# Autodesk Inventor assembly: 041.5
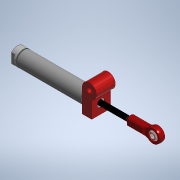
[picture p0: Inventor's stored thumbnail of the model, 180x180]
Saved by Autodesk Inventor 2020 (Build 240168000, 168)
## iProperties
Part Number: 041.5
Catalog Web Link: www.cadenas.de
Description: Original Line Standard Air Cylinders-Standard Air Cylinders
Vendor: BIMBA
Document SubType Name: Assembly
Designer: partserver
Manufacturer: BIMBA
Mass: 46.5963 g
Surface Area: 273.014 cm^2
Volume: 39.6045 cm^3
Density: 1.17654 g/cm^3
Category: PARTsolutions
Company: BIMBA
PSOL_IDENT_0: {$CADENAS_DATA\23d-libs\bimba\bimba_brand\bimba_imperial\bimba_full_line\original_line_cylinders\sta
PSOL_IDENT_1: ndard_air_cylinders\standard_air_cylinder_asmtab.prj},318 {VTYP=3D},{STYP=ASSTAB},{NB=041.5},{LINA=0
PSOL_IDENT_2: 41.5},{NN=Original Line Standard Air Cylinders},{DATE=19.01.2022 10:19:38},{GEOMDATE=11.11.2021 07:3
PSOL_IDENT_3: 1:43},{VERSION=},{LINEID=50},{WBVAR=STROKE,ACTING,MNT,DER,NR,BM,CO,OO,VO,M,EE,EEL,K,Q,Y,G,T,HL,B,H,S
PSOL_IDENT_4: ER,SR,NT,W,STPT1,STPT2,STPT3,STPT4,MB,PB,PRC,TB,MN},{WBNUMERIC=STROKE,EEL}  {NB=041.5},{LINA=041.5},
PSOL_IDENT_5: {KT=DUMMY},{PN=041.5},{PNC=041.5},{PNA=(NO ACCESSORIES)},{PNAHELP=},{DASH=},{BORE1=0.75000000},{BORE=
PSOL_IDENT_6: 3/4\" (04)},{BOREPN=04},{STROKE=1.500},{STROKEALG=[0.011:50/0.001]},{STROKE1=1.500},{ACTING=},{ACTIN
PSOL_IDENT_7: GALG= '' , 'Single Acting' , 'R' , 'Reverse Single Acting (R)' , 'D' , 'Double Acting (D)' },{ACTING
PSOL_IDENT_8: PN=},{MNT=},{MNTALG= '' , 'Front Nose Mounting' , 'P' , 'Rear Pivot Mounting (P)' , 'BF' , 'Front Bl
PSOL_IDENT_9: ock Mounting (BF)' , 'BR' , 'Rear Block Mounting for Vertical Positioning (BR)' , 'BFT' , 'Front Blo
PSOL_IDENT_10: ck Trunnion Mounting (BFT)' , 'BRT' , 'Rear Block Trunnion Mounting (BRT)' , 'A' , 'Double End Mount
PSOL_IDENT_11: ing with Brackets and Adjustable Stroke (A)' , 'AP' , 'Rear Pivot Mounting with Adjustable Stroke (A
PSOL_IDENT_12: P)' },{TYPE=},{MNTPN=},{DER=},{DERALG= '' , 'N/A' },{NR=},{NRALG= '' , 'Round (Standard)' , 'NR' , '
PSOL_IDENT_13: Non-rotating - Hexagon Rod' },{NRPN=},{BM=},{BMALG= '' , 'Without Built-in Midget 3-Way Solenoid Ope
PSOL_IDENT_14: rated Valve' , 'LS' , 'With LS Series Solenoid Valve [LS]' },{BMPN=},{CO=},{COALG= '' , 'N/A' },{OO=
PSOL_IDENT_15: },{OOALG= '', 'N/A' },{OOPN=},{VO=Z},{VOALG= 'Z' , 'N/A' },{VOPN=},{OOVOPN=},{M=},{MALG= '', 'Withou
PSOL_IDENT_16: t Magnet', 'M', 'With Magnet' },{EE=},{EEL=0.000},{EEMAX=48.5000},{EEALG= '', 'Without Extra Extensi
PSOL_IDENT_17: on', 'EE', 'With Extra Extension' },{EELALG=0},{EEPN=},{EEPN1=0.000},{K=},{KALG= '' , 'N/A' },{KPN=}
PSOL_IDENT_18: ,{Q=},{QALG= '' , 'Standard Port' , 'Q' , 'Side Port' },{QPN=},{Y=},{YALG= '' , 'N/A' },{YPN=},{YCON=
PSOL_IDENT_19: },{F=},{FALG= '', 'Non-Coated (Standard)', 'F', 'Molycoated' },{FPN=},{G=},{GPN=},{GPN99=},{T=},{TAL
PSOL_IDENT_20: G= '' , 'Standard -20° to 200°F (-29° to 95°C)' , 'N' , 'Low Temperature' , 'V' , 'High Temperature'
PSOL_IDENT_21: },{NPN=},{VPN=},{HL=},{HLALG= '' , 'N/A' },{B=},{BALG= '', 'W/out Bumpers' , 'B' , 'W/ Bumpers' },{
PSOL_IDENT_22: BPN=},{H=},{HALG= '', 'W/ Standard Spring (Relaxed 3 lbs./Compressed 6 lbs.)', 'H', 'W/ Heavy Spring
PSOL_IDENT_23: (Relaxed 4 lbs./Compressed 10 lbs.)' },{HPN=},{SER=},{SERALG= '' , 'N/A' },{SR=C},{SRALG= 'C' , 'St
PSOL_IDENT_24: andard Blackened Carbon Steel' , 'SR' , 'Stainless Steel [SR]' },{SRPN=},{SRCON=1},{NT=},{NTPN=},{W=
PSOL_IDENT_25: },{WALG= '' , 'N/A' },{WPN=},{E=},{EALG= '' , 'Standard Seals/Lube' , 'E' , 'Non-Lube Seals/Lube' },
PSOL_IDENT_26: {EPN=},{ST=},{STALG= '' , 'N/A' },{STPT1=},{STPT1ALG= '' , 'N/A' },{STPT2=},{STPT2ALG= '' , 'N/A' },
PSOL_IDENT_27: {STPT3=},{STPT3ALG= '' , 'N/A' },{STPT4=},{STPT4ALG= '' , 'N/A' },{STPN=},{MB=},{MBALG= '' , 'Withou
PSOL_IDENT_28: t Mounting Bracket' , 'F,D-226' , 'D-226 (front)' },{MBPN=},{MBPNALL=D-226},{MBPNALLREAR=},{PB=},{PB
PSOL_IDENT_29: ALG= '' , 'N/A' },{PBPN=},{PBPNALL=},{PRC=},{PRCALG= '' , 'W/out Pivot Rod Clevis' , 'F,D-166-3' , '
PSOL_IDENT_30: D-166-3 (front)' },{PRCPN=},{PRCPNALL=D-166-3},{TB=},{TBALG= '' , 'N/A' },{TBPN=},{TBPNALL=},{MN=},{
PSOL_IDENT_31: MNALG= '' , 'N/A' },{MNPN=},{MNCONF=},{MNCONR=},{TLEN=3.4460},{FRAC=4.3800},{RGCON=},{RGDACCON=},{RH
PSOL_IDENT_32: CON=},{RHCON1=},{RHCONON=1},{RHACCON=},{FNUTCON=1},{RNUTCON=0},{FNUTPN=D-98},{RNUTPN=},{FNUTTRANS=0.
PSOL_IDENT_33: 0000},{RNUTTRANS=0.0000},{VHOLECON=2},{A1=0.8750},{A1N=0.8750},{A1P=1.5940},{A1B=1.5940},{A4=0.3130}
PSOL_IDENT_34: ,{A4N=0.3130},{A4P=0.2525},{A5=0.0300},{A1H=0.531},{A1NH=0.5310},{A1PH=1.5940},{A1BH=1.0940},{A1SH=1
PSOL_IDENT_35: .2190},{A2H=0.2190},{A2NH=0.2190},{LENGTH=1.5000},{LENGTH1=1.5000},{LENGTH2=3.0300},{MUL=2.5350},{MU
PSOL_IDENT_36: L11=2.5350},{MUL22=4.035},{MUL33=2.5350},{MUL2=1.6900},{MUL211=1.6900},{MUL222=2.6900},{MUL233=1.690
PSOL_IDENT_37: 0},{SSS=3.0000},{RGLEN=0.5920},{RHLEN=0.3420},{SSS1=2.0000},{A13=1.3120},{DIF=0.0000},{G5=0.6250},{O
PSOL_IDENT_38: N=0},{SSADD=0.0000},{BADD=0.0000},{MADD=0.0000},{NVADD=0.0000},{TRACKL=3.1560},{TRACKCON=D-74168},{T
PSOL_IDENT_39: RIMCON=0},{TRIMCON1=0},{PINCON=},{FSPACE=0.5679},{SPACE=0.0589},{TEXT=0.1031},{S1=1.0000},{D1=0.8050
PSOL_IDENT_40: },{D1N=0.8050},{D1B=0.8625},{D1P=0.8325},{FA=0.750},{RA=0.0000},{PPATH=standard_air_cylinder_asmtpl.
PSOL_IDENT_41: prj},{MATALGHTML=<b>Standard Original Line:</b><dl><dt>Rod:</dt><dd>- Stainless Steel</dd><dd>&nbsp;
PSOL_IDENT_42: &nbsp;(5/16 9/16 Bores)</dd><dd>- High Strength Carbon Steel</dd><dd>&nbsp;&nbsp;(3/4 3 Bore)</dd><d
PSOL_IDENT_43: d>- Stainless Steel</dd><dd>&nbsp;&nbsp;(X style DXP/DX/DXDE)</dd><dt>Bearings:</dt><dd>- Sintered B
PSOL_IDENT_44: ronze</dd><dt>Body:</dt><dd>- 304 Stainless Steel</dd><dt>End Caps:</dt><dd>- Aluminum</dd><dt>Seals
PSOL_IDENT_45: :</dt><dd>- Buna N</dd></dl>},{ASSCFGPRA=04},{MBPNA=},{MNPNA=},{PRCPNA=},{ASSOPTACC=STPT4},{A=4.38},
PSOL_IDENT_46: {HADD=0.0000},{WFL=0.25},{QADD=0.000},{QADD1=0.440},{TEST=1.0000},{MNTB=},{STDNUTF=1},{STDNUTR=0},{S
PSOL_IDENT_47: TRK2D=0},{X2D=2},{STROKESW=1.500},{EESW=0.000},{FCD=0},{BCD=0},{RCD=0},{CUSTADD=0.500},{FT=1/4-28 UN
PSOL_IDENT_48: F-2A},{FT1=1/4-28 UNF-2A},{FT2=5/8-18 UNF-2A},{PORT=1/8 NPT},{FT11=1/2-20 UNF-2A},{FT12=5/8-18 UNF-2
PSOL_IDENT_49: A},{B1=}
NB: 041.5
NN: Original Line Standard Air Cylinders
NT: Threaded (Standard)
NBSYN: $PNC.
LINA: 041.5
CATALOG: Bimba Products
PN: 041.5
PNA: (NO ACCESSORIES)
BORE: 3/4" (04)
STROKE: 1.5
ACTING: Single [Standard]
MNT: Front Nose
DER: N/A
NR: Round (Standard)
BM: Without Built-in Midget 3-Way Solenoid Operated Valve
CO: N/A
OO: N/A
VO: N/A
M: Without Magnet
EE: Without Extra Extension
EEL: 0
K: N/A
Q: Standard Port
Y: N/A
G: Standard Lube
T: Standard -20° to 200°F (-29° to 95°C)
HL: N/A
B: W/out Bumpers
H: W/ Standard Spring (Relaxed 3 lbs./Compressed 6 lbs.)
SER: N/A
SR: Standard Blackened Carbon Steel
W: N/A
STPT1: N/A
STPT2: N/A
STPT3: N/A
STPT4: N/A
MB: Without Mounting Bracket
PB: N/A
PRC: W/out Pivot Rod Clevis
TB: N/A
MN: N/A
A: 4.38
SUPPLIER: BIMBA
ARTICLENO: 041.5
BOMINFO: 041.5
CREATOR: CADENAS GmbH
Title: 041.5
Author: Cadenas PARTsolutions
Comments: Standard Air Cylinders
## Documents named in this file (8)
- T:\EIT\2022 Rapid React\COMMON PARTS\AIR CYLINDERS\BIMBA_0415\AIS2020\041_5.iam
- T:\EIT\2022 Rapid React\COMMON PARTS\AIR CYLINDERS\BIMBA_0415\AIS2020\041_5C0000000_0_dummy.ipt
- T:\EIT\2022 Rapid React\COMMON PARTS\AIR CYLINDERS\BIMBA_0415\AIS2020\04000-0_rod_guide.ipt
- T:\EIT\2022 Rapid React\COMMON PARTS\AIR CYLINDERS\BIMBA_0415\AIS2020\04-3_4462C.ipt
- T:\EIT\2022 Rapid React\COMMON PARTS\AIR CYLINDERS\BIMBA_0415\AIS2020\040000_rear_head.ipt
- T:\EIT\2022 Rapid React\COMMON PARTS\AIR CYLINDERS\BIMBA_0415\AIS2020\C-041_50000_rod.ipt
- T:\EIT\2022 Rapid React\COMMON PARTS\AIR CYLINDERS\TieRod End\60685K321_PTFE-LINED ALUMINUM BALL JOINT ROD END.ipt
- T:\EIT\2022 Rapid React\SHOOTER\SH-ACM-001.ipt
## Components (7 placed, 7 different names)
1. 041_5C0000000_0_dummy:1
2. 04000-0_rod_guide:1 — Insert:1, Insert:3
3. 04-3_4462C:1
4. 040000_rear_head:1 — Angle:1
5. C-041_50000_rod:1 — Insert:1, Insert:2
6. 60685K321_PTFE-LINED ALUMINUM BALL JOINT ROD END:1 — Insert:2, Angle:1, Angle:2
7. SH-ACM-001:1 — Insert:3, Angle:2
## Relationships (5: Insert 3, Angle 2)
- Insert:1 (38.1 mm): 04000-0_rod_guide:1 ↔ C-041_50000_rod:1
- Insert:2 (3.175 mm): C-041_50000_rod:1 ↔ 60685K321_PTFE-LINED ALUMINUM BALL JOINT ROD END:1
- Angle:1 (0 deg): 040000_rear_head:1 ↔ 60685K321_PTFE-LINED ALUMINUM BALL JOINT ROD END:1
- Insert:3: 04000-0_rod_guide:1 ↔ SH-ACM-001:1
- Angle:2 (0 deg): 60685K321_PTFE-LINED ALUMINUM BALL JOINT ROD END:1 ↔ SH-ACM-001:1
